# Autodesk Inventor assembly: FULL SWERVE DRIVE ASSEMBLY!  5!
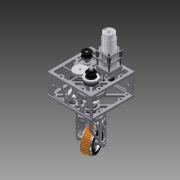
[picture p0: Inventor's stored thumbnail of the model, 180x180]
Saved by Autodesk Inventor 2012 (Build 160160000, 160)
## iProperties
Created: 2013-01-01
Part Number: FULL SWERVE DRIVE ASSEMBLY!  5!
Document SubType Name: Assembly
Designer: Bryce
Author: Bryce
## Documents named in this file (16)
- C:\Users\Bryce\Dropbox\Inventor Design Project Files\Independent Swerves\Inventor 2012\FULL SWERVE DRIVE ASSEMBLY!  5!.iam
- C:\Users\Bryce\Dropbox\Inventor Design Project Files\Independent Swerves\Inventor 2012\collar bearing systom.ipt
- C:\Users\Bryce\Dropbox\Inventor Design Project Files\Independent Swerves\Imported Components\CIM Motor.iam
- C:\Users\Bryce\Dropbox\Inventor Design Project Files\Independent Swerves\Inventor 2012\turn encoder assembly.iam
- C:\Users\Bryce\Dropbox\Inventor Design Project Files\Independent Swerves\Imported Components\Imported Components\48-5m09-6a5\48-5m09-6a5.ipt
- C:\Users\Bryce\Dropbox\Inventor Design Project Files\Independent Swerves\Inventor 2012\frame assembly 2.iam
- C:\Users\Bryce\Dropbox\Inventor Design Project Files\Independent Swerves\Imported Components\15T plastick sprocket .375.ipt
- C:\Users\Bryce\Dropbox\Inventor Design Project Files\Independent Swerves\Imported Components\15T plastick sprocket 8mm.ipt
- C:\Users\Bryce\Dropbox\Inventor Design Project Files\Independent Swerves\Imported Components\15T plastick sprocket .375 threaded.ipt
- C:\Users\Bryce\Dropbox\Inventor Design Project Files\Independent Swerves\Inventor 2012\sprocket hub adaptor.ipt
- C:\Users\Bryce\Dropbox\Inventor Design Project Files\Independent Swerves\Inventor 2012\tensioning wedge.ipt
- C:\Users\Bryce\Dropbox\Inventor Design Project Files\Independent Swerves\Imported Components\BD Gearbox and Bracket Assy 4.iam
- C:\Users\Bryce\Dropbox\Inventor Design Project Files\Independent Swerves\Inventor 2012\Lower box main assembly 5.iam
- C:\Users\Bryce\Dropbox\Inventor Design Project Files\Independent Swerves\Inventor 2012\upper gearbox frame 4.ipt
- C:\Users\Bryce\Dropbox\Inventor Design Project Files\Independent Swerves\Imported Components\encoder gear small.ipt
- C:\Users\Bryce\Dropbox\Inventor Design Project Files\Independent Swerves\Imported Components\encoder gear turn small.ipt
## Components (18 placed, 15 different names)
1. upper gearbox frame 4:1 — Mate:1, Mate:2, Mate:3, Mate:4, Mate:11, Mate:15, Mate:16, Mate:17, Mate:18, Angle:2, Mate:24, Mate:25, Mate:26, Mate:40, Mate:41, Flush:15, Flush:16, Mate:50, Mate:51, Mate:52, Mate:53, Mate:54, Mate:55, Mate:56, Mate:58
2. collar bearing systom:1 — Mate:1, Mate:2
3. collar bearing systom:2 — Mate:3, Mate:4, Mate:59, Flush:18
4. BD Gearbox and Bracket Assy 4:1 [sub-assembly] — Mate:40, Mate:41, Mate:46, Mate:47, Mate:54, Mate:58
5. CIM Motor:1 [sub-assembly] — Mate:11, Mate:42, Mate:55, Mate:56
6. turn encoder assembly:1 [sub-assembly] — Mate:17, Mate:18, Angle:1, Angle:2, Rotation:3, Rotation:4
7. turn encoder assembly:2 [sub-assembly] — Mate:15, Mate:16, Angle:1, Rotation:2
8. encoder gear turn small:1 — Rotation:3, Rotation:4, Mate:61, Flush:19
9. 48-5m09-6a5:1 — Flush:17, Mate:63, Flush:21
10. frame assembly 2:1 [sub-assembly] — Mate:24, Mate:25, Mate:26
11. 15T plastick sprocket .375 threaded:1 — Mate:46, Mate:47, Flush:17
12. 15T plastick sprocket 8mm:1 — Mate:42, Mate:48, Mate:49, Flush:13, Flush:14, Rotation:7, Mate:57
13. encoder gear small:1 — Rotation:2, Mate:44, Rotation:6, Mate:60
14. 15T plastick sprocket .375:1 — Mate:44, Rotation:6, Flush:14, Rotation:7, Mate:57, Mate:62, Flush:20
15. sprocket hub adaptor:1 — Mate:48, Mate:49, Flush:13
16. tensioning wedge:1 — Flush:15, Mate:50, Mate:52
17. tensioning wedge:2 — Flush:16, Mate:51, Mate:53
18. Lower box main assembly 5:1 [sub-assembly] — Mate:59, Flush:18, Mate:60, Mate:61, Flush:19, Mate:62, Flush:20, Mate:63, Flush:21
## Relationships (53: Mate 34, Flush 11, RelateRotation 6, Angle 2)
- Mate:1: upper gearbox frame 4:1 ↔ collar bearing systom:1
- Mate:2: upper gearbox frame 4:1 ↔ collar bearing systom:1
- Mate:3: upper gearbox frame 4:1 ↔ collar bearing systom:2
- Mate:4: upper gearbox frame 4:1 ↔ collar bearing systom:2
- Mate:11: upper gearbox frame 4:1 ↔ CIM Motor:1
- Mate:15: upper gearbox frame 4:1 ↔ turn encoder assembly:2
- Mate:16: upper gearbox frame 4:1 ↔ turn encoder assembly:2
- Mate:17: upper gearbox frame 4:1 ↔ turn encoder assembly:1
- Mate:18: upper gearbox frame 4:1 ↔ turn encoder assembly:1
- [Flush]: turn encoder assembly:1 ↔ encoder gear turn small:1
- Angle:1 (0 deg): turn encoder assembly:1 ↔ turn encoder assembly:2
- Angle:2 (0 deg): upper gearbox frame 4:1 ↔ turn encoder assembly:1
- Mate:24: upper gearbox frame 4:1 ↔ frame assembly 2:1
- Mate:25: upper gearbox frame 4:1 ↔ frame assembly 2:1
- Mate:26: upper gearbox frame 4:1 ↔ frame assembly 2:1
- [Flush]: turn encoder assembly:2 ↔ encoder gear small:1
- Rotation:2 [RelateRotation] (1 ul): turn encoder assembly:2 ↔ encoder gear small:1
- Rotation:3 [RelateRotation] (1 ul): turn encoder assembly:1 ↔ encoder gear turn small:1
- Rotation:4 [RelateRotation] (1 ul): turn encoder assembly:1 ↔ encoder gear turn small:1
- Mate:40 (3.175 mm): upper gearbox frame 4:1 ↔ BD Gearbox and Bracket Assy 4:1
- Mate:41 (3.175 mm): upper gearbox frame 4:1 ↔ BD Gearbox and Bracket Assy 4:1
- [RelateRotation] (0.3333 ul): 48-5m09-6a5:1 ↔ 15T plastick sprocket .375 threaded:1
- Mate:42: CIM Motor:1 ↔ 15T plastick sprocket 8mm:1
- Mate:44: encoder gear small:1 ↔ 15T plastick sprocket .375:1
- Rotation:6 [RelateRotation] (1 ul): encoder gear small:1 ↔ 15T plastick sprocket .375:1
- Mate:46: BD Gearbox and Bracket Assy 4:1 ↔ 15T plastick sprocket .375 threaded:1
- Mate:47 (3.175 mm): BD Gearbox and Bracket Assy 4:1 ↔ 15T plastick sprocket .375 threaded:1
- Mate:48: 15T plastick sprocket 8mm:1 ↔ sprocket hub adaptor:1
- Mate:49: 15T plastick sprocket 8mm:1 ↔ sprocket hub adaptor:1
- Flush:13: 15T plastick sprocket 8mm:1 ↔ sprocket hub adaptor:1
- Flush:14: 15T plastick sprocket 8mm:1 ↔ 15T plastick sprocket .375:1
- Flush:15 (-6.35 mm): upper gearbox frame 4:1 ↔ tensioning wedge:1
- Flush:16 (-6.35 mm): upper gearbox frame 4:1 ↔ tensioning wedge:2
- Mate:50: upper gearbox frame 4:1 ↔ tensioning wedge:1
- Mate:51: upper gearbox frame 4:1 ↔ tensioning wedge:2
- Mate:52: upper gearbox frame 4:1 ↔ tensioning wedge:1
- Mate:53: upper gearbox frame 4:1 ↔ tensioning wedge:2
- Flush:17 (0.254 mm): 48-5m09-6a5:1 ↔ 15T plastick sprocket .375 threaded:1
- Mate:54: upper gearbox frame 4:1 ↔ BD Gearbox and Bracket Assy 4:1
- Rotation:7 [RelateRotation] (1 ul): 15T plastick sprocket 8mm:1 ↔ 15T plastick sprocket .375:1
- Mate:55 (2.54 mm): upper gearbox frame 4:1 ↔ CIM Motor:1
- Mate:56 (2.54 mm): upper gearbox frame 4:1 ↔ CIM Motor:1
- Mate:57 (88.9 mm): 15T plastick sprocket 8mm:1 ↔ 15T plastick sprocket .375:1
- Mate:58 (9.525 mm): upper gearbox frame 4:1 ↔ BD Gearbox and Bracket Assy 4:1
- Mate:59: collar bearing systom:2 ↔ Lower box main assembly 5:1
- Flush:18 (-1.27 mm): collar bearing systom:2 ↔ Lower box main assembly 5:1
- Mate:60: encoder gear small:1 ↔ Lower box main assembly 5:1
- Mate:61: encoder gear turn small:1 ↔ Lower box main assembly 5:1
- Flush:19: encoder gear turn small:1 ↔ Lower box main assembly 5:1
- Mate:62: 15T plastick sprocket .375:1 ↔ Lower box main assembly 5:1
- Flush:20: 15T plastick sprocket .375:1 ↔ Lower box main assembly 5:1
- Mate:63: 48-5m09-6a5:1 ↔ Lower box main assembly 5:1
- Flush:21: 48-5m09-6a5:1 ↔ Lower box main assembly 5:1
